# Autodesk Inventor assembly: Infineon-STP_PG-TO247-3-901-P-v01_00-EN
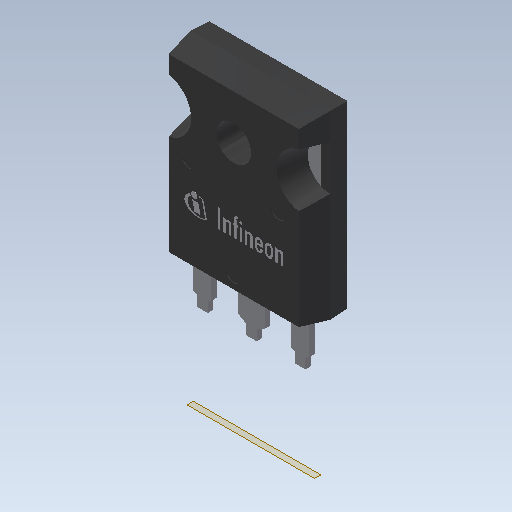
[picture p0: Inventor's stored thumbnail of the model, 512x512]
Saved by Autodesk Inventor 2020 (Build 240168000, 168)
## iProperties
Created: 2017-12-13
Part Number: Infineon-STP_PG-TO247-3-901-P-v01_00-EN
Document SubType Name: Assembly
Designer: jg_ma
Sending System: Autodesk Inventor 2014
Preprocessor: ST-DEVELOPER v15.2
Title: C:\Users\mdsaid\Documents\Project\03 IR Integration\POL\20171212\PG-TO247-3-901\3D_Model\PG-TO247-3-901\PG-TO247-3-901.stp
Author: mdsaid
## Documents named in this file (8)
- C:\Users\Acer\Documents\ssl-mechanics\V2.1(LARC2019)\Inventor\sec_floor\Components\KickerBoard\Infineon-STP_PG-TO247-3-901-P-v01_00-EN\Infineon-STP_PG-TO247-3-901-P-v01_00-EN.iam
- C:\Users\Acer\Documents\ssl-mechanics\V2.1(LARC2019)\Inventor\sec_floor\Components\KickerBoard\Infineon-STP_PG-TO247-3-901-P-v01_00-EN\PG-TO247-3-901_LOWER_MOLD.ipt
- C:\Users\Acer\Documents\ssl-mechanics\V2.1(LARC2019)\Inventor\sec_floor\Components\KickerBoard\Infineon-STP_PG-TO247-3-901-P-v01_00-EN\PG-TO247-3-901_UPPER_MOLD.ipt
- C:\Users\Acer\Documents\ssl-mechanics\V2.1(LARC2019)\Inventor\sec_floor\Components\KickerBoard\Infineon-STP_PG-TO247-3-901-P-v01_00-EN\PG-TO247-3-901_EXPOSED_PAD_1.ipt
- C:\Users\Acer\Documents\ssl-mechanics\V2.1(LARC2019)\Inventor\sec_floor\Components\KickerBoard\Infineon-STP_PG-TO247-3-901-P-v01_00-EN\PG-TO247-3-901_EXPOSED_PAD_2.ipt
- C:\Users\Acer\Documents\ssl-mechanics\V2.1(LARC2019)\Inventor\sec_floor\Components\KickerBoard\Infineon-STP_PG-TO247-3-901-P-v01_00-EN\PG-TO247-3-901_EXPOSED_LEAD_1.ipt
- C:\Users\Acer\Documents\ssl-mechanics\V2.1(LARC2019)\Inventor\sec_floor\Components\KickerBoard\Infineon-STP_PG-TO247-3-901-P-v01_00-EN\PG-TO247-3-901_EXPOSED_LEAD_2.ipt
- C:\Users\Acer\Documents\ssl-mechanics\V2.1(LARC2019)\Inventor\sec_floor\Components\KickerBoard\Infineon-STP_PG-TO247-3-901-P-v01_00-EN\PG-TO247-3-901_LOGO.ipt
## Components (8 placed, 8 different names)
1. PG-TO247-3-901_LOWER_MOLD:1
2. PG-TO247-3-901_UPPER_MOLD:1
3. PG-TO247-3-901_EXPOSED_PAD_1:1
4. PG-TO247-3-901_EXPOSED_PAD_2:1
5. PG-TO247-3-901_EXPOSED_LEAD_1 — Mate:1, Mate:2
6. PG-TO247-3-901_EXPOSED_LEAD_2
7. PG-TO247-3-901_EXPOSED_LEAD_3 — Mate:3
8. PG-TO247-3-901_LOGO:1
## Relationships (3: Mate 3)
- Mate:1: PG-TO247-3-901_EXPOSED_LEAD_1
- Mate:2: PG-TO247-3-901_EXPOSED_LEAD_1
- Mate:3: PG-TO247-3-901_EXPOSED_LEAD_3
